# Autodesk Inventor assembly: main assem
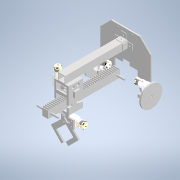
[picture p0: Inventor's stored thumbnail of the model, 180x180]
Saved by Autodesk Inventor 2020.1 (Build 241239000, 239)
## iProperties
Created: 2019-11-07
Part Number: main assem
Document SubType Name: Assembly
Designer: amirs
Author: amirs
## Documents named in this file (6)
- C:\Users\amirs\OneDrive - UC San Diego\college\freshman year\MAE 3\robot\main assem.iam
- C:\Users\amirs\Downloads\grabber assembly.iam
- C:\Users\amirs\Downloads\base.iam
- C:\Users\amirs\OneDrive - UC San Diego\college\freshman year\MAE 3\robot\metal tube piece.ipt
- C:\Users\amirs\OneDrive - UC San Diego\college\freshman year\MAE 3\robot\l-bracket.ipt
- C:\Users\amirs\Downloads\rack and pinion.iam
## Components (7 placed, 5 different names)
1. grabber assembly:1 [sub-assembly] — Mate:11, Flush:13, Flush:5, Flush:14, Mate:13
2. base:1 [sub-assembly] — Mate:7, Flush:5, Mate:12
3. metal tube piece:1 — Mate:1, Mate:2, Flush:1, Mate:3, Mate:4, Flush:2, Mate:5, Mate:6, Flush:3, Mate:8, Mate:9, Mate:10, Mate:12
4. l-bracket:1 — Mate:5, Mate:6, Flush:3, Mate:7
5. l-bracket:2 — Mate:3, Mate:4, Flush:2
6. l-bracket:3 — Mate:1, Mate:2, Flush:1
7. rack and pinion:1 [sub-assembly] — Mate:8, Mate:9, Mate:10, Mate:11, Flush:13, Flush:14, Mate:13
## Relationships (19: Mate 13, Flush 6)
- Mate:1: metal tube piece:1 ↔ l-bracket:3
- Mate:2: metal tube piece:1 ↔ l-bracket:3
- Flush:1: metal tube piece:1 ↔ l-bracket:3
- Mate:3: metal tube piece:1 ↔ l-bracket:2
- Mate:4: metal tube piece:1 ↔ l-bracket:2
- Flush:2: metal tube piece:1 ↔ l-bracket:2
- Mate:5: metal tube piece:1 ↔ l-bracket:1
- Mate:6: metal tube piece:1 ↔ l-bracket:1
- Flush:3: metal tube piece:1 ↔ l-bracket:1
- Mate:7 (5.08 mm): base:1 ↔ l-bracket:1
- Mate:8: metal tube piece:1 ↔ rack and pinion:1
- Mate:9: metal tube piece:1 ↔ rack and pinion:1
- Mate:10: metal tube piece:1 ↔ rack and pinion:1
- Mate:11: grabber assembly:1 ↔ rack and pinion:1
- Flush:13 (177.8 mm): grabber assembly:1 ↔ rack and pinion:1
- Flush:5: grabber assembly:1 ↔ base:1
- Flush:14: grabber assembly:1 ↔ rack and pinion:1
- Mate:12: base:1 ↔ metal tube piece:1
- Mate:13: grabber assembly:1 ↔ rack and pinion:1
